# Autodesk Inventor assembly: Chess Board
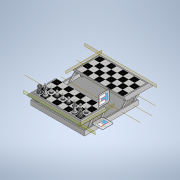
[picture p0: Inventor's stored thumbnail of the model, 180x180]
Saved by Autodesk Inventor 2022 (Build 260153000, 153)
## iProperties
Created: 2022-04-03
Part Number: Chess Board
Document SubType Name: Assembly
Designer: Nick
Author: Nick
## Documents named in this file (9)
- Y:\Projects\Chess_Board\Chess Board.iam
- Y:\Projects\Chess_Board\Top Base.ipt
- Y:\Projects\Chess_Board\Bottom Base.ipt
- Y:\Projects\Chess_Board\Board Pattern.iam
- Y:\Projects\Chess_Board\Angle Bracket.ipt
- Y:\Projects\Chess_Board\Linkage.ipt
- Y:\Projects\Chess_Board\Pieces\Pawn.ipt
- Y:\Projects\Chess_Board\Pieces\Rook.ipt
- Y:\Projects\Chess_Board\Pieces\Knight.ipt
## Components (33 placed, 8 different names)
1. Top Base:1 — Mate:9, Mate:10, Mate:15, Mate:22, Mate:23, Mate:24
2. Top Base:2 — Mate:11, Mate:12, Mate:13, Mate:14, Mate:26, Mate:29, Mate:30, Mate:34
3. Bottom Base:1 — Mate:1, Mate:2, Mate:3, Mate:4, Mate:10, Mate:11, Mate:17, Mate:25, Mate:27, Mate:28, Mate:31, Mate:32, Mate:33, Angle:5
4. Board Pattern:1 [sub-assembly] — Mate:22, Mate:23, Mate:24
5. Board Pattern:2 [sub-assembly] — Mate:12, Mate:13, Mate:14, Mate:35, Mate:36, Mate:37, Mate:38, Mate:39, Mate:40, Mate:41, Mate:42, Mate:43, Mate:44, Mate:45, Mate:46, Mate:47, Mate:48, Mate:49, Mate:50, Mate:51, Mate:52, Mate:53, Mate:54, Mate:55, Mate:56, Mate:57, Mate:58
6. Angle Bracket:1 — Insert:1, Flush:2, Mate:18
7. Angle Bracket:2 — Flush:1, Mate:5, Mate:6, Mate:19
8. Angle Bracket:3 — Insert:2, Flush:2, Mate:19
9. Angle Bracket:4 — Flush:1, Mate:7, Mate:8, Mate:9, Mate:15, Mate:18
10. Linkage:1 — Mate:1, Mate:2, Angle:1, Mate:5, Mate:6, Mate:20
11. Linkage:3 — Mate:3, Mate:4, Angle:1, Mate:7, Mate:8, Mate:21
12. Linkage:4 — Insert:2, Flush:7, Mate:17, Mate:20
13. Linkage:5 — Insert:1, Flush:7, Mate:21
14. Angle Bracket:5 — Mate:30, Mate:34
15. Angle Bracket:6
16. Linkage:6 — Flush:6, Mate:32
17. Linkage:7 — Flush:6, Mate:31, Mate:33
18. Angle Bracket:7
19. Angle Bracket:8 — Mate:26, Mate:29
20. Linkage:8 — Flush:5, Mate:25, Mate:27
21. Linkage:9 — Flush:5, Mate:28
22. Pawn:1 — Mate:35, Mate:36
23. Pawn:2 — Mate:40, Mate:47
24. Pawn:3 — Mate:41, Mate:50
25. Pawn:4 — Mate:37, Mate:46
26. Pawn:5 — Mate:39, Mate:45
27. Pawn:6 — Mate:38, Mate:44
28. Pawn:7 — Mate:43, Mate:48
29. Pawn:8 — Mate:42, Mate:49
30. Rook:1 — Mate:52, Mate:53
31. Rook:2 — Mate:51, Mate:54
32. Knight:1 — Mate:56, Mate:58, Angle:5, Angle:6
33. Knight:2 — Mate:55, Mate:57, Angle:6
## Relationships (76: Mate 57, Flush 7, Angle 6, Insert 6)
- Mate:1: Bottom Base:1 ↔ Linkage:1
- Mate:2: Bottom Base:1 ↔ Linkage:1
- Mate:3: Bottom Base:1 ↔ Linkage:3
- Mate:4: Bottom Base:1 ↔ Linkage:3
- Angle:1 (180 deg): Linkage:1 ↔ Linkage:3
- Flush:1: Angle Bracket:2 ↔ Angle Bracket:4
- Mate:5: Angle Bracket:2 ↔ Linkage:1
- Mate:6: Angle Bracket:2 ↔ Linkage:1
- Mate:7: Angle Bracket:4 ↔ Linkage:3
- Mate:8: Angle Bracket:4 ↔ Linkage:3
- Mate:9: Top Base:1 ↔ Angle Bracket:4
- Mate:10: Top Base:1 ↔ Bottom Base:1
- Mate:11: Top Base:2 ↔ Bottom Base:1
- Mate:12: Top Base:2 ↔ Board Pattern:2
- Mate:13: Top Base:2 ↔ Board Pattern:2
- Mate:14: Top Base:2 ↔ Board Pattern:2
- Mate:15 (73.025 mm): Top Base:1 ↔ Angle Bracket:4
- [Angle] (180 deg): Linkage:4 ↔ Linkage:5
- Insert:1: Angle Bracket:1 ↔ Linkage:5
- Insert:2: Angle Bracket:3 ↔ Linkage:4
- Flush:2: Angle Bracket:1 ↔ Angle Bracket:3
- [Angle] (180 deg): Linkage:6 ↔ Linkage:7
- [Insert]: Angle Bracket:5 ↔ Linkage:7
- [Insert]: Angle Bracket:6 ↔ Linkage:6
- [Flush]: Angle Bracket:5 ↔ Angle Bracket:6
- [Angle] (180 deg): Linkage:8 ↔ Linkage:9
- [Insert]: Angle Bracket:7 ↔ Linkage:9
- [Insert]: Angle Bracket:8 ↔ Linkage:8
- [Flush]: Angle Bracket:7 ↔ Angle Bracket:8
- Flush:5: Linkage:8 ↔ Linkage:9
- Flush:6: Linkage:6 ↔ Linkage:7
- Flush:7: Linkage:4 ↔ Linkage:5
- Mate:17: Bottom Base:1 ↔ Linkage:4
- Mate:18: Angle Bracket:1 ↔ Angle Bracket:4
- Mate:19: Angle Bracket:2 ↔ Angle Bracket:3
- Mate:20: Linkage:1 ↔ Linkage:4
- Mate:21: Linkage:3 ↔ Linkage:5
- Mate:22: Top Base:1 ↔ Board Pattern:1
- Mate:23: Top Base:1 ↔ Board Pattern:1
- Mate:24: Top Base:1 ↔ Board Pattern:1
- Mate:25: Bottom Base:1 ↔ Linkage:8
- Mate:26: Top Base:2 ↔ Angle Bracket:8
- Mate:27: Bottom Base:1 ↔ Linkage:8
- Mate:28: Bottom Base:1 ↔ Linkage:9
- Mate:29 (73.025 mm): Top Base:2 ↔ Angle Bracket:8
- Mate:30: Top Base:2 ↔ Angle Bracket:5
- Mate:31: Bottom Base:1 ↔ Linkage:7
- Mate:32: Bottom Base:1 ↔ Linkage:6
- Mate:33: Bottom Base:1 ↔ Linkage:7
- Mate:34 (73.025 mm): Top Base:2 ↔ Angle Bracket:5
- Mate:35: Board Pattern:2 ↔ Pawn:1
- Mate:36: Board Pattern:2 ↔ Pawn:1
- Mate:37: Board Pattern:2 ↔ Pawn:4
- Mate:38: Board Pattern:2 ↔ Pawn:6
- Mate:39: Board Pattern:2 ↔ Pawn:5
- Mate:40: Board Pattern:2 ↔ Pawn:2
- Mate:41: Board Pattern:2 ↔ Pawn:3
- Mate:42: Board Pattern:2 ↔ Pawn:8
- Mate:43: Board Pattern:2 ↔ Pawn:7
- Mate:44: Board Pattern:2 ↔ Pawn:6
- Mate:45: Board Pattern:2 ↔ Pawn:5
- Mate:46: Board Pattern:2 ↔ Pawn:4
- Mate:47: Board Pattern:2 ↔ Pawn:2
- Mate:48: Board Pattern:2 ↔ Pawn:7
- Mate:49: Board Pattern:2 ↔ Pawn:8
- Mate:50: Board Pattern:2 ↔ Pawn:3
- Mate:51: Board Pattern:2 ↔ Rook:2
- Mate:52: Board Pattern:2 ↔ Rook:1
- Mate:53: Board Pattern:2 ↔ Rook:1
- Mate:54: Board Pattern:2 ↔ Rook:2
- Mate:55: Board Pattern:2 ↔ Knight:2
- Mate:56: Board Pattern:2 ↔ Knight:1
- Mate:57: Board Pattern:2 ↔ Knight:2
- Mate:58: Board Pattern:2 ↔ Knight:1
- Angle:5 (180 deg): Bottom Base:1 ↔ Knight:1
- Angle:6 (0 deg): Knight:1 ↔ Knight:2
## Named parameters: d91_d77 = 180 deg, d95_d91_d77 = 180 deg, d96_d92 = 0 mm, d97_d93 = 0 mm, d98_d94 = 0 mm, d99_d91_d77 = 180 deg, d100_d92 = 0 mm, d101_d93 = 0 mm, d102_d94 = 0 mm
